# Autodesk Inventor assembly: Topassembly
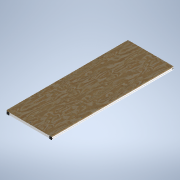
[picture p0: Inventor's stored thumbnail of the model, 180x180]
Saved by Autodesk Inventor 2020.2 (Build 242310000, 310)
## iProperties
Created: 2020-07-25
Part Number: Topassembly
Document SubType Name: Assembly
Designer: JK
Author: JK
## Documents named in this file (8)
- C:\Users\JK\Documents\Inventor\Mesa\Topassembly.iam
- C:\Users\JK\Documents\Inventor\Mesa\30x30x1500.ipt
- C:\Users\JK\Documents\Inventor\Mesa\30x30x500.ipt
- C:\Users\JK\Documents\Inventor\Mesa\Top.ipt
- C:\Users\JK\Documents\Inventor\Mesa\boltnuttopassembly.iam
- C:\Users\JK\Documents\Inventor\Mesa\Cornerassembly.iam
- C:\Users\JK\Documents\Inventor\Mesa\boltnuttopassembly_MIR.iam
- C:\Users\JK\Documents\Inventor\Mesa\3030_endCap v4.ipt
## Components (25 placed, 7 different names)
1. 30x30x1500:1 — Flush:2, Mate:3, Flush:5, Flush:6, Flush:7, Mate:13, Flush:11, Mate:14, Mate:20, Mate:22, Flush:13, Flush:14, Flush:19, Flush:20
2. 30x30x1500:2 — Mate:1, Flush:1, Mate:2, Flush:3, Mate:7, Mate:8, Flush:9, Mate:11, Mate:19, Mate:21, Flush:15, Flush:16, Flush:17, Flush:18
3. 30x30x500:1 — Mate:1, Flush:1, Flush:2, Flush:6, Flush:8, Mate:10, Flush:10, Mate:12
4. 30x30x500:2 — Mate:2, Mate:3, Flush:3, Flush:5, Mate:9, Mate:15, Flush:12, Angle:2
5. Top:1 — Flush:7, Flush:8, Mate:4, Angle:1, Mate:7, Mate:16, Mate:17, Mate:18
6. Cornerassembly:1 [sub-assembly] — Mate:8, Flush:9, Mate:9
7. Cornerassembly:2 [sub-assembly] — Mate:14, Mate:15, Flush:12
8. Cornerassembly:3 [sub-assembly] — Mate:12, Mate:13, Flush:11
9. Cornerassembly:4 [sub-assembly] — Mate:10, Flush:10, Mate:11
10. boltnuttopassembly:11 [sub-assembly] — Mate:16, Mate:17, Angle:2
11. boltnuttopassembly_MIR:1 [sub-assembly]
12. 3030_endCap v4:1 — Mate:22, Flush:13, Flush:14
13. 3030_endCap v4:2 — Mate:19, Flush:17, Flush:18
14. 3030_endCap v4:3 — Mate:20, Flush:19, Flush:20
15. 3030_endCap v4:4 — Mate:21, Flush:15, Flush:16
16. boltnuttopassembly:1 [sub-assembly] — Mate:4, Angle:1, Mate:18
17. boltnuttopassembly:12 [sub-assembly]
18. boltnuttopassembly:13 [sub-assembly]
19. boltnuttopassembly:14 [sub-assembly]
20. boltnuttopassembly:15 [sub-assembly]
21. boltnuttopassembly:16 [sub-assembly]
22. boltnuttopassembly:17 [sub-assembly]
23. boltnuttopassembly:18 [sub-assembly]
24. boltnuttopassembly:19 [sub-assembly]
25. boltnuttopassembly:20 [sub-assembly]
## Component patterns: (10 elements, first: boltnuttopassembly:1)
## Relationships (41: Mate 20, Flush 19, Angle 2)
- Mate:1: 30x30x1500:2 ↔ 30x30x500:1
- Flush:1: 30x30x1500:2 ↔ 30x30x500:1
- Flush:2: 30x30x1500:1 ↔ 30x30x500:1
- Mate:2: 30x30x1500:2 ↔ 30x30x500:2
- Mate:3: 30x30x1500:1 ↔ 30x30x500:2
- Flush:3: 30x30x1500:2 ↔ 30x30x500:2
- Flush:5: 30x30x1500:1 ↔ 30x30x500:2
- Flush:6: 30x30x1500:1 ↔ 30x30x500:1
- Flush:7: 30x30x1500:1 ↔ Top:1
- Flush:8: 30x30x500:1 ↔ Top:1
- Mate:4: Top:1 ↔ boltnuttopassembly:1
- Angle:1 (0 deg): Top:1 ↔ boltnuttopassembly:1
- Mate:7: 30x30x1500:2 ↔ Top:1
- Mate:8: 30x30x1500:2 ↔ Cornerassembly:1
- Flush:9 (0.5 mm): 30x30x1500:2 ↔ Cornerassembly:1
- Mate:9: 30x30x500:2 ↔ Cornerassembly:1
- Mate:10: 30x30x500:1 ↔ Cornerassembly:4
- Flush:10 (0.5 mm): 30x30x500:1 ↔ Cornerassembly:4
- Mate:11: 30x30x1500:2 ↔ Cornerassembly:4
- Mate:12: 30x30x500:1 ↔ Cornerassembly:3
- Mate:13: 30x30x1500:1 ↔ Cornerassembly:3
- Flush:11 (0.5 mm): 30x30x1500:1 ↔ Cornerassembly:3
- Mate:14: 30x30x1500:1 ↔ Cornerassembly:2
- Mate:15: 30x30x500:2 ↔ Cornerassembly:2
- Flush:12 (0.5 mm): 30x30x500:2 ↔ Cornerassembly:2
- Mate:16: Top:1 ↔ boltnuttopassembly:11
- Mate:17: Top:1 ↔ boltnuttopassembly:11
- Angle:2 (0 deg): 30x30x500:2 ↔ boltnuttopassembly:11
- Mate:18: Top:1 ↔ boltnuttopassembly:1
- Mate:19: 30x30x1500:2 ↔ 3030_endCap v4:2
- Mate:20: 30x30x1500:1 ↔ 3030_endCap v4:3
- Mate:21: 30x30x1500:2 ↔ 3030_endCap v4:4
- Mate:22: 30x30x1500:1 ↔ 3030_endCap v4:1
- Flush:13: 30x30x1500:1 ↔ 3030_endCap v4:1
- Flush:14: 30x30x1500:1 ↔ 3030_endCap v4:1
- Flush:15: 30x30x1500:2 ↔ 3030_endCap v4:4
- Flush:16: 30x30x1500:2 ↔ 3030_endCap v4:4
- Flush:17: 30x30x1500:2 ↔ 3030_endCap v4:2
- Flush:18: 30x30x1500:2 ↔ 3030_endCap v4:2
- Flush:19: 30x30x1500:1 ↔ 3030_endCap v4:3
- Flush:20: 30x30x1500:1 ↔ 3030_endCap v4:3
